# Autodesk Inventor assembly: main
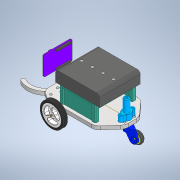
[picture p0: Inventor's stored thumbnail of the model, 180x180]
Saved by Autodesk Inventor 2020 (Build 240168000, 168)
## iProperties
Created: 2020-11-02
Part Number: main
Document SubType Name: Assembly
Designer: alnwlsn
Author: alnwlsn
## Documents named in this file (20)
- C:\Users\alnwlsn\lizard-sync\3d-printer-cad\part-files\wilson-products\esp-rov\main.iam
- C:\Users\alnwlsn\lizard-sync\3d-printer-cad\part-files\wilson-products\esp-rov\n20.ipt
- C:\Users\alnwlsn\lizard-sync\3d-printer-cad\part-files\wilson-products\esp-rov\drwheel.ipt
- C:\Users\alnwlsn\lizard-sync\3d-printer-cad\part-files\wilson-products\esp-rov\idl-tire.ipt
- C:\Users\alnwlsn\lizard-sync\3d-printer-cad\part-files\wilson-products\esp-rov\idl-bearing.ipt
- C:\Users\alnwlsn\lizard-sync\3d-printer-cad\part-files\wilson-products\esp-rov\caster-h.ipt
- C:\Users\alnwlsn\lizard-sync\3d-printer-cad\part-files\wilson-products\esp-rov\chassis.ipt
- C:\Users\alnwlsn\lizard-sync\3d-printer-cad\part-files\wilson-products\esp-rov\motor-clamp.ipt
- C:\Users\alnwlsn\lizard-sync\3d-printer-cad\part-files\wilson-products\esp-rov\4aa-holder.ipt
- C:\Users\alnwlsn\lizard-sync\3d-printer-cad\part-files\wilson-products\esp-rov\esp32-cam-sp.ipt
- C:\Users\alnwlsn\lizard-sync\3d-printer-cad\part-files\wilson-products\esp-rov\caster-bng.ipt
- C:\Users\alnwlsn\lizard-sync\3d-printer-cad\part-files\wilson-products\esp-rov\9g-servo.ipt
- C:\Users\alnwlsn\lizard-sync\3d-printer-cad\part-files\wilson-products\esp-rov\servo-horn-b.ipt
- C:\Users\alnwlsn\lizard-sync\3d-printer-cad\part-files\wilson-products\esp-rov\caster-spacer.ipt
- C:\Users\alnwlsn\lizard-sync\3d-printer-cad\part-files\wilson-products\esp-rov\claw-w.ipt
- C:\Users\alnwlsn\lizard-sync\3d-printer-cad\part-files\wilson-products\esp-rov\claw-w_MIR1.ipt
- C:\Users\alnwlsn\lizard-sync\3d-printer-cad\part-files\wilson-products\esp-rov\batt-standoff.ipt
- C:\Users\alnwlsn\lizard-sync\3d-printer-cad\part-files\wilson-products\esp-rov\ff.ipt
- C:\Users\alnwlsn\lizard-sync\3d-printer-cad\part-files\wilson-products\esp-rov\f3.ipt
- C:\Users\alnwlsn\lizard-sync\3d-printer-cad\part-files\wilson-products\esp-rov\ff2.ipt
## Components (22 placed, 19 different names)
1. n20:1 — Mate:1, Mate:2, Flush:1, Flush:2, Mate:12
2. n20:2 — Mate:3, Mate:4, Flush:1, Flush:2, Mate:9, Mate:10, Mate:11, Mate:14, Angle:1
3. drwheel:1 — Mate:1, Mate:2, Tangent:1
4. drwheel:2 — Mate:3, Mate:4
5. idl-tire:1 — Mate:5, Mate:6
6. idl-bearing:1 — Mate:5, Mate:6, Mate:7, Mate:8
7. caster-h:1 — Mate:7, Mate:8, Angle:3, Mate:26, Mate:27
8. chassis:1 — Mate:9, Mate:10, Mate:11, Mate:12, Mate:13, Angle:2, Mate:24, Mate:25, Angle:4, Mate:30, Mate:31, Mate:32, Mate:40, Mate:41, Mate:44, Mate:50, Mate:54, Angle:6
9. motor-clamp:1 — Mate:13, Mate:14, Angle:1, Mate:15, Flush:4
10. motor-clamp:2 — Mate:15, Flush:4
11. esp32-cam-sp:1
12. 4aa-holder:1 — Mate:53
13. caster-bng:1 — Mate:24, Mate:25, Angle:4, Mate:26, Mate:28, Mate:29
14. 9g-servo:1 — Mate:22, Mate:23, Mate:30, Mate:31, Mate:32
15. servo-horn-b:2 — Mate:22, Mate:23, Mate:62
16. caster-spacer:1 — Mate:27, Mate:28, Mate:29
17. claw-w:1 — Mate:40, Mate:41, Flush:5, Mate:63
18. claw-w_MIR1:1 — Mate:44, Flush:5, Mate:67
19. batt-standoff:1 — Mate:50, Mate:53, Mate:54, Angle:6
20. ff:1 — Mate:62, Mate:63, Mate:64, Mate:65
21. f3:1 — Mate:64, Mate:65, Mate:66
22. ff2:1 — Mate:66, Mate:67
## Relationships (49: Mate 38, Flush 5, Angle 5, Tangent 1)
- Mate:1: n20:1 ↔ drwheel:1
- Mate:2: n20:1 ↔ drwheel:1
- Mate:3: n20:2 ↔ drwheel:2
- Mate:4: n20:2 ↔ drwheel:2
- Flush:1: n20:1 ↔ n20:2
- Flush:2: n20:1 ↔ n20:2
- Mate:5: idl-tire:1 ↔ idl-bearing:1
- Mate:6: idl-tire:1 ↔ idl-bearing:1
- Mate:7: idl-bearing:1 ↔ caster-h:1
- Mate:8: idl-bearing:1 ↔ caster-h:1
- Mate:9: n20:2 ↔ chassis:1
- Mate:10: n20:2 ↔ chassis:1
- Mate:11: n20:2 ↔ chassis:1
- Mate:12: n20:1 ↔ chassis:1
- Mate:13: chassis:1 ↔ motor-clamp:1
- Mate:14: n20:2 ↔ motor-clamp:1
- Angle:1 (0 deg): n20:2 ↔ motor-clamp:1
- Flush:3
- Tangent:1: drwheel:1
- Angle:2 (0 deg): chassis:1
- Angle:3 (0 deg): caster-h:1
- Mate:15: motor-clamp:1 ↔ motor-clamp:2
- Flush:4: motor-clamp:1 ↔ motor-clamp:2
- Mate:22: 9g-servo:1 ↔ servo-horn-b:2
- Mate:23: 9g-servo:1 ↔ servo-horn-b:2
- Mate:24: chassis:1 ↔ caster-bng:1
- Mate:25: chassis:1 ↔ caster-bng:1
- Angle:4 (0 deg): chassis:1 ↔ caster-bng:1
- Mate:26: caster-h:1 ↔ caster-bng:1
- Mate:27: caster-h:1 ↔ caster-spacer:1
- Mate:28: caster-bng:1 ↔ caster-spacer:1
- Mate:29: caster-bng:1 ↔ caster-spacer:1
- Mate:30 (0.1 mm): chassis:1 ↔ 9g-servo:1
- Mate:31: chassis:1 ↔ 9g-servo:1
- Mate:32: chassis:1 ↔ 9g-servo:1
- Mate:40: chassis:1 ↔ claw-w:1
- Mate:41: chassis:1 ↔ claw-w:1
- Mate:44: chassis:1 ↔ claw-w_MIR1:1
- Flush:5: claw-w:1 ↔ claw-w_MIR1:1
- Mate:50: chassis:1 ↔ batt-standoff:1
- Mate:53: 4aa-holder:1 ↔ batt-standoff:1
- Mate:54: chassis:1 ↔ batt-standoff:1
- Angle:6 (0 deg): chassis:1 ↔ batt-standoff:1
- Mate:62: servo-horn-b:2 ↔ ff:1
- Mate:63: claw-w:1 ↔ ff:1
- Mate:64: ff:1 ↔ f3:1
- Mate:65: ff:1 ↔ f3:1
- Mate:66: f3:1 ↔ ff2:1
- Mate:67: claw-w_MIR1:1 ↔ ff2:1
